# Autodesk Inventor assembly: Head
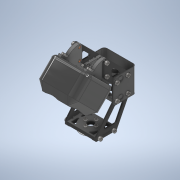
[picture p0: Inventor's stored thumbnail of the model, 180x180]
Saved by Autodesk Inventor 2022.3 (Build 263350000, 350)
## iProperties
Created: 2021-12-31
Part Number: Head
Document SubType Name: Assembly
Designer: Masato Kubotera
Mass: 92.9564 g
Surface Area: 535.434 cm^2
Volume: 94.1049 cm^3
Density: 0.987795 g/cm^3
Author: Masato Kubotera
## Documents named in this file (14)
- C:\Users\Masato\Documents\Inventor\CIT Brains\SUSTAINA-OP - mod\UpperBody\Head\Head.iam
- C:\Users\Masato\Documents\Inventor\CIT Brains\SUSTAINA-OP - mod\UpperBody\Head\CameraUnit_e-CAM50_CUNX.iam
- C:\Users\Masato\Documents\Inventor\CIT Brains\SUSTAINA-OP - mod\UpperBody\Head\Camera_side_frame.ipt
- C:\Users\Masato\Documents\Inventor\CIT Brains\SUSTAINA-OP - mod\ReadyMade\InsertNut\UD-43040.ipt
- C:\Users\Masato\Documents\Inventor\CIT Brains\SUSTAINA-OP - mod\UpperBody\Head\Head_side_frame.ipt
- C:\Users\Masato\Documents\Inventor\CIT Brains\SUSTAINA-OP - mod\ReadyMade\Screw\UC-0306.ipt
- C:\Users\Masato\Documents\Inventor\CIT Brains\SUSTAINA-OP - mod\UpperBody\UpperBody_horn_frame.ipt
- C:\Users\Masato\Documents\Inventor\CIT Brains\SUSTAINA-OP - mod\ReadyMade\InsertNut\IRU-304S.ipt
- C:\Users\Masato\Documents\Inventor\CIT Brains\SUSTAINA-OP - mod\ReadyMade\Washer\TT-2532-20.ipt
- C:\Users\Masato\Documents\Inventor\CIT Brains\SUSTAINA-OP - mod\ReadyMade\Screw\UC-2610.ipt
- C:\Users\Masato\Documents\Inventor\CIT Brains\SUSTAINA-OP - mod\UpperBody\Head\Head_diagonal.ipt
- C:\Users\Masato\Documents\Inventor\CIT Brains\SUSTAINA-OP - mod\ReadyMade\Bush\L3040-8110TB.ipt
- C:\Users\Masato\Documents\Inventor\CIT Brains\SUSTAINA-OP - mod\ReadyMade\Screw\UC-0308.ipt
- C:\Users\Masato\Documents\Inventor\CIT Brains\SUSTAINA-OP - mod\UpperBody\Head\Head_back_cloth.ipt
## Components (54 placed, 13 different names)
1. CameraUnit_e-CAM50_CUNX:1 [sub-assembly] — 挿入:1, 挿入:2, 挿入:3, 挿入:4
2. TT-2532-20:1 — 挿入:29
3. L3040-8110TB:4 — 挿入:81, 挿入:85
4. L3040-8110TB:3 — 挿入:80, 挿入:84
5. L3040-8110TB:2 — 挿入:79, 挿入:83, 挿入:87
6. L3040-8110TB:1 — 挿入:78, 挿入:82, 挿入:86
7. Head_back_cloth:1 — 挿入:86, 挿入:87
8. Camera_side_frame:1 — 挿入:1, 挿入:2, 挿入:5, 挿入:6, 挿入:88, 挿入:89
9. Camera_side_frame:2 — 挿入:3, 挿入:4, 挿入:7, 挿入:8, 挿入:90, 挿入:91
10. Head_side_frame:1 — 挿入:13, 挿入:14, 挿入:17, 挿入:18, 挿入:25, 挿入:26, 挿入:34, 挿入:35, 挿入:46, 挿入:47, 挿入:52, 挿入:53, 挿入:54, 挿入:58, 挿入:78, 挿入:79
11. Head_side_frame:2 — 挿入:15, 挿入:16, 挿入:19, 挿入:20, 挿入:27, 挿入:28, 挿入:36, 挿入:37, 挿入:48, 挿入:49, 挿入:50, 挿入:51, 挿入:56, 挿入:60, 挿入:80, 挿入:81
12. Head_diagonal:1 — 挿入:38, 挿入:39, 挿入:40, 挿入:41
13. Head_diagonal:2 — 挿入:42, 挿入:43, 挿入:44, 挿入:45
14. UpperBody_horn_frame:1 — 挿入:21, 挿入:22, 挿入:23, 挿入:24, 挿入:29, 挿入:30, 挿入:31, 挿入:32, 挿入:33, メイト:1, メイト:2, メイト:3
15. UC-0308:4 — 挿入:85
16. UC-0308:3 — 挿入:84
17. UC-0308:2 — 挿入:82
18. UC-0308:1 — 挿入:83
19. UC-0308:5 — 挿入:88
20. UC-0308:6 — 挿入:90
21. UC-0308:7 — 挿入:89
22. UC-0308:8 — 挿入:91
23. UC-0306:1 — 挿入:17
24. UC-0306:2 — 挿入:18
25. UC-0306:3 — 挿入:19
26. UC-0306:4 — 挿入:20
27. UC-0306:5 — 挿入:34
28. UC-0306:6 — 挿入:35
29. UC-0306:7 — 挿入:36
30. UC-0306:8 — 挿入:37
31. UC-0306:9 — 挿入:54
32. UC-0306:11 — 挿入:56
33. UC-0306:13 — 挿入:58
34. UC-0306:15 — 挿入:60
35. UC-2610:1 — 挿入:30
36. UC-2610:2 — 挿入:31
37. UC-2610:3 — 挿入:32
38. UC-2610:4 — 挿入:33
39. UD-43040:1 — 挿入:5, 挿入:13
40. UD-43040:2 — 挿入:6, 挿入:14
41. UD-43040:3 — 挿入:7, 挿入:15
42. UD-43040:4 — 挿入:8, 挿入:16
43. IRU-304S:1 — 挿入:21, 挿入:25
44. IRU-304S:2 — 挿入:22, 挿入:26
45. IRU-304S:3 — 挿入:23, 挿入:28
46. IRU-304S:4 — 挿入:24, 挿入:27
47. IRU-304S:5 — 挿入:38, 挿入:46
48. IRU-304S:6 — 挿入:39, 挿入:47
49. IRU-304S:7 — 挿入:40, 挿入:48
50. IRU-304S:8 — 挿入:41, 挿入:49
51. IRU-304S:9 — 挿入:42, 挿入:53
52. IRU-304S:10 — 挿入:43, 挿入:52
53. IRU-304S:11 — 挿入:44, 挿入:50
54. IRU-304S:12 — 挿入:45, 挿入:51
## Relationships (70: Insert 67, Mate 3)
- 挿入:1 [Insert]: CameraUnit_e-CAM50_CUNX:1 ↔ Camera_side_frame:1
- 挿入:2 [Insert]: CameraUnit_e-CAM50_CUNX:1 ↔ Camera_side_frame:1
- 挿入:3 [Insert]: CameraUnit_e-CAM50_CUNX:1 ↔ Camera_side_frame:2
- 挿入:4 [Insert]: CameraUnit_e-CAM50_CUNX:1 ↔ Camera_side_frame:2
- 挿入:5 [Insert]: Camera_side_frame:1 ↔ UD-43040:1
- 挿入:6 [Insert]: Camera_side_frame:1 ↔ UD-43040:2
- 挿入:7 [Insert]: Camera_side_frame:2 ↔ UD-43040:3
- 挿入:8 [Insert]: Camera_side_frame:2 ↔ UD-43040:4
- 挿入:13 [Insert]: Head_side_frame:1 ↔ UD-43040:1
- 挿入:14 [Insert]: Head_side_frame:1 ↔ UD-43040:2
- 挿入:15 [Insert]: Head_side_frame:2 ↔ UD-43040:3
- 挿入:16 [Insert]: Head_side_frame:2 ↔ UD-43040:4
- 挿入:17 [Insert]: Head_side_frame:1 ↔ UC-0306:1
- 挿入:18 [Insert]: Head_side_frame:1 ↔ UC-0306:2
- 挿入:19 [Insert]: Head_side_frame:2 ↔ UC-0306:3
- 挿入:20 [Insert]: Head_side_frame:2 ↔ UC-0306:4
- 挿入:21 [Insert]: UpperBody_horn_frame:1 ↔ IRU-304S:1
- 挿入:22 [Insert]: UpperBody_horn_frame:1 ↔ IRU-304S:2
- 挿入:23 [Insert]: UpperBody_horn_frame:1 ↔ IRU-304S:3
- 挿入:24 [Insert]: UpperBody_horn_frame:1 ↔ IRU-304S:4
- 挿入:25 [Insert]: Head_side_frame:1 ↔ IRU-304S:1
- 挿入:26 [Insert]: Head_side_frame:1 ↔ IRU-304S:2
- 挿入:27 [Insert]: Head_side_frame:2 ↔ IRU-304S:4
- 挿入:28 [Insert]: Head_side_frame:2 ↔ IRU-304S:3
- 挿入:29 [Insert]: TT-2532-20:1 ↔ UpperBody_horn_frame:1
- 挿入:30 [Insert]: UpperBody_horn_frame:1 ↔ UC-2610:1
- 挿入:31 [Insert]: UpperBody_horn_frame:1 ↔ UC-2610:2
- 挿入:32 [Insert]: UpperBody_horn_frame:1 ↔ UC-2610:3
- 挿入:33 [Insert]: UpperBody_horn_frame:1 ↔ UC-2610:4
- 挿入:34 [Insert]: Head_side_frame:1 ↔ UC-0306:5
- 挿入:35 [Insert]: Head_side_frame:1 ↔ UC-0306:6
- 挿入:36 [Insert]: Head_side_frame:2 ↔ UC-0306:7
- 挿入:37 [Insert]: Head_side_frame:2 ↔ UC-0306:8
- 挿入:38 [Insert]: Head_diagonal:1 ↔ IRU-304S:5
- 挿入:39 [Insert]: Head_diagonal:1 ↔ IRU-304S:6
- 挿入:40 [Insert]: Head_diagonal:1 ↔ IRU-304S:7
- 挿入:41 [Insert]: Head_diagonal:1 ↔ IRU-304S:8
- 挿入:42 [Insert]: Head_diagonal:2 ↔ IRU-304S:9
- 挿入:43 [Insert]: Head_diagonal:2 ↔ IRU-304S:10
- 挿入:44 [Insert]: Head_diagonal:2 ↔ IRU-304S:11
- 挿入:45 [Insert]: Head_diagonal:2 ↔ IRU-304S:12
- 挿入:46 [Insert]: Head_side_frame:1 ↔ IRU-304S:5
- 挿入:47 [Insert]: Head_side_frame:1 ↔ IRU-304S:6
- 挿入:48 [Insert]: Head_side_frame:2 ↔ IRU-304S:7
- 挿入:49 [Insert]: Head_side_frame:2 ↔ IRU-304S:8
- 挿入:50 [Insert]: Head_side_frame:2 ↔ IRU-304S:11
- 挿入:51 [Insert]: Head_side_frame:2 ↔ IRU-304S:12
- 挿入:52 [Insert]: Head_side_frame:1 ↔ IRU-304S:10
- 挿入:53 [Insert]: Head_side_frame:1 ↔ IRU-304S:9
- 挿入:54 [Insert]: Head_side_frame:1 ↔ UC-0306:9
- 挿入:56 [Insert]: Head_side_frame:2 ↔ UC-0306:11
- 挿入:58 [Insert]: Head_side_frame:1 ↔ UC-0306:13
- 挿入:60 [Insert]: Head_side_frame:2 ↔ UC-0306:15
- メイト:1 [Mate]: UpperBody_horn_frame:1
- メイト:2 [Mate]: UpperBody_horn_frame:1
- メイト:3 [Mate]: UpperBody_horn_frame:1
- 挿入:78 [Insert]: L3040-8110TB:1 ↔ Head_side_frame:1
- 挿入:79 [Insert]: L3040-8110TB:2 ↔ Head_side_frame:1
- 挿入:80 [Insert]: L3040-8110TB:3 ↔ Head_side_frame:2
- 挿入:81 [Insert]: L3040-8110TB:4 ↔ Head_side_frame:2
- 挿入:82 [Insert]: L3040-8110TB:1 ↔ UC-0308:2
- 挿入:83 [Insert]: L3040-8110TB:2 ↔ UC-0308:1
- 挿入:84 [Insert]: L3040-8110TB:3 ↔ UC-0308:3
- 挿入:85 [Insert]: L3040-8110TB:4 ↔ UC-0308:4
- 挿入:86 [Insert]: L3040-8110TB:1 ↔ Head_back_cloth:1
- 挿入:87 [Insert]: L3040-8110TB:2 ↔ Head_back_cloth:1
- 挿入:88 [Insert]: Camera_side_frame:1 ↔ UC-0308:5
- 挿入:89 [Insert]: Camera_side_frame:1 ↔ UC-0308:7
- 挿入:90 [Insert]: Camera_side_frame:2 ↔ UC-0308:6
- 挿入:91 [Insert]: Camera_side_frame:2 ↔ UC-0308:8
